# Autodesk Inventor assembly: Claw
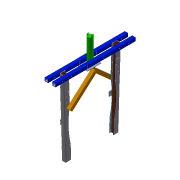
[picture p0: Inventor's stored thumbnail of the model, 180x180]
Saved by Autodesk Inventor 2015 (Build 190159000, 159)
## iProperties
Created: 2015-01-13
Part Number: Claw
Document SubType Name: Assembly
Designer: Collin_2
Author: Collin_2
## Documents named in this file (11)
- C:\Users\Tanner\Documents\GitHub\FIRST-Team-1719-CAD-Team\2015 Robot CAD\Devices\Claw\Claw.iam
- C:\Users\Tanner\Documents\GitHub\FIRST-Team-1719-CAD-Team\2015 Robot CAD\Devices\Claw\Claw - Base.ipt
- C:\Users\Tanner\Documents\GitHub\FIRST-Team-1719-CAD-Team\2015 Robot CAD\Devices\Claw\PC3.5-P1.ipt
- C:\Users\Tanner\Documents\GitHub\FIRST-Team-1719-CAD-Team\2015 Robot CAD\Devices\Claw\PC3.5-ROD.ipt
- C:\Users\Tanner\Documents\GitHub\FIRST-Team-1719-CAD-Team\2015 Robot CAD\Devices\Claw\Claw - Arm - Top (R).ipt
- C:\Users\Tanner\Documents\GitHub\FIRST-Team-1719-CAD-Team\2015 Robot CAD\Devices\Claw\Claw - Arm - Bottom (R).ipt
- C:\Users\Tanner\Documents\GitHub\FIRST-Team-1719-CAD-Team\2015 Robot CAD\Devices\Claw\Claw - Arm - Middle.ipt
- C:\Users\Tanner\Documents\GitHub\FIRST-Team-1719-CAD-Team\2015 Robot CAD\Devices\Claw\Yarm.ipt
- C:\Users\Tanner\Documents\GitHub\FIRST-Team-1719-CAD-Team\2015 Robot CAD\Devices\Claw\Claw - Arm - Plate.ipt
- C:\Users\Tanner\Documents\GitHub\FIRST-Team-1719-CAD-Team\2015 Robot CAD\Devices\Claw\Claw - L bracket.ipt
- C:\Users\Tanner\Documents\GitHub\FIRST-Team-1719-CAD-Team\2015 Robot CAD\Devices\Claw\Claw - Arm - Plate 2.ipt
## Components (17 placed, 10 different names)
1. Claw - Base:1 — Mate:18, Mate:19, Mate:20, Mate:21, Tangent:2, Flush:8, Mate:52, Flush:9, Flush:10
2. PC3.5-P1:1 — Mate:15, Mate:16, Tangent:2, Mate:53
3. PC3.5-ROD:1 — Mate:15, Mate:16, Mate:37, Mate:55
4. Claw - Arm - Top (R):1 — Mate:20, Mate:21, Mate:26, Mate:27, Mate:38, Insert:4, Mate:50, Insert:6
5. Claw - Arm - Top (R):2 — Mate:23, Mate:24, Mate:31, Mate:35, Flush:5, Insert:3, Angle:1
6. Claw - Arm - Bottom (R):1 — Mate:18, Mate:19, Mate:23, Mate:24, Mate:41, Insert:2, Flush:7, Mate:51, Insert:5
7. Claw - Arm - Bottom (R):2 — Mate:26, Mate:27, Flush:4, Mate:47, Flush:6, Insert:1, Mate:48, Mate:49, Mate:54, Angle:2
8. Claw - Arm - Middle:1 — Mate:31, Mate:41, Flush:5, Mate:51
9. Claw - Arm - Middle:2 — Flush:4, Mate:48, Mate:49, Mate:50
10. Yarm:1 — Mate:35, Mate:37, Mate:40, Insert:3
11. Yarm:2 — Mate:38, Mate:40, Insert:4, Mate:55
12. Claw - Arm - Plate:1 — Mate:47, Flush:6, Insert:1
13. Claw - Arm - Plate:2 — Insert:2, Flush:7
14. Claw - L bracket:1 — Flush:8, Mate:52, Mate:53
15. Claw - Base:2 — Mate:54, Flush:9, Flush:10
16. Claw - Arm - Plate 2:1 — Insert:5, Angle:1
17. Claw - Arm - Plate 2:2 — Insert:6, Angle:2
## Relationships (41: Mate 25, Flush 7, Insert 6, Angle 2, Tangent 1)
- Mate:15: PC3.5-P1:1 ↔ PC3.5-ROD:1
- Mate:16: PC3.5-P1:1 ↔ PC3.5-ROD:1
- Mate:18: Claw - Base:1 ↔ Claw - Arm - Bottom (R):1
- Mate:19: Claw - Base:1 ↔ Claw - Arm - Bottom (R):1
- Mate:20: Claw - Base:1 ↔ Claw - Arm - Top (R):1
- Mate:21: Claw - Base:1 ↔ Claw - Arm - Top (R):1
- Mate:23: Claw - Arm - Top (R):2 ↔ Claw - Arm - Bottom (R):1
- Mate:24: Claw - Arm - Top (R):2 ↔ Claw - Arm - Bottom (R):1
- Mate:26: Claw - Arm - Top (R):1 ↔ Claw - Arm - Bottom (R):2
- Mate:27: Claw - Arm - Top (R):1 ↔ Claw - Arm - Bottom (R):2
- Mate:31: Claw - Arm - Top (R):2 ↔ Claw - Arm - Middle:1
- Mate:35: Claw - Arm - Top (R):2 ↔ Yarm:1
- Mate:37: PC3.5-ROD:1 ↔ Yarm:1
- Mate:38: Claw - Arm - Top (R):1 ↔ Yarm:2
- Mate:40: Yarm:1 ↔ Yarm:2
- Tangent:2 (285.75 mm): Claw - Base:1 ↔ PC3.5-P1:1
- Mate:41: Claw - Arm - Bottom (R):1 ↔ Claw - Arm - Middle:1
- Flush:4: Claw - Arm - Bottom (R):2 ↔ Claw - Arm - Middle:2
- Flush:5: Claw - Arm - Top (R):2 ↔ Claw - Arm - Middle:1
- Mate:47: Claw - Arm - Bottom (R):2 ↔ Claw - Arm - Plate:1
- Flush:6: Claw - Arm - Bottom (R):2 ↔ Claw - Arm - Plate:1
- Insert:1: Claw - Arm - Bottom (R):2 ↔ Claw - Arm - Plate:1
- Insert:2: Claw - Arm - Bottom (R):1 ↔ Claw - Arm - Plate:2
- Flush:7: Claw - Arm - Bottom (R):1 ↔ Claw - Arm - Plate:2
- Mate:48: Claw - Arm - Bottom (R):2 ↔ Claw - Arm - Middle:2
- Mate:49: Claw - Arm - Bottom (R):2 ↔ Claw - Arm - Middle:2
- Insert:3: Claw - Arm - Top (R):2 ↔ Yarm:1
- Insert:4: Claw - Arm - Top (R):1 ↔ Yarm:2
- Mate:50: Claw - Arm - Top (R):1 ↔ Claw - Arm - Middle:2
- Mate:51: Claw - Arm - Bottom (R):1 ↔ Claw - Arm - Middle:1
- Flush:8: Claw - Base:1 ↔ Claw - L bracket:1
- Mate:52: Claw - Base:1 ↔ Claw - L bracket:1
- Mate:53: PC3.5-P1:1 ↔ Claw - L bracket:1
- Mate:54: Claw - Arm - Bottom (R):2 ↔ Claw - Base:2
- Flush:9: Claw - Base:1 ↔ Claw - Base:2
- Flush:10: Claw - Base:1 ↔ Claw - Base:2
- Mate:55: PC3.5-ROD:1 ↔ Yarm:2
- Insert:5: Claw - Arm - Bottom (R):1 ↔ Claw - Arm - Plate 2:1
- Insert:6: Claw - Arm - Top (R):1 ↔ Claw - Arm - Plate 2:2
- Angle:1 (0 deg): Claw - Arm - Top (R):2 ↔ Claw - Arm - Plate 2:1
- Angle:2 (0 deg): Claw - Arm - Bottom (R):2 ↔ Claw - Arm - Plate 2:2
